# Autodesk Inventor assembly: Handle_ASAP3
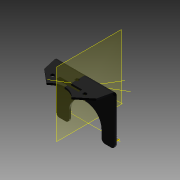
[picture p0: Inventor's stored thumbnail of the model, 180x180]
Saved by Autodesk Inventor 2011 SP2 (Build 150309200, 309)
## iProperties
Created: 2013-03-14
Part Number: Handle_ASAP3
Document SubType Name: Assembly
Designer: sungwook
Author: sungwook
## Documents named in this file (4)
- C:\Users\sungwook\Documents\Inventor\Micron22_top_adj_02082013\Parts\ASAP\Handle_ASAP3.iam
- C:\Users\sungwook\Documents\Inventor\Micron22_top_adj_02082013\Parts\ASAP\ASAP_Handle_Fixture_New3.ipt
- C:\Users\sungwook\Documents\Inventor\Micron22_top_adj_02082013\Parts\ASAP\LED2.ipt
- C:\Users\sungwook\Documents\Inventor\Micron22_top_adj_02082013\Parts\ASAP\LED2_MIR3.ipt
## Components (4 placed, 3 different names)
1. ASAP_Handle_Fixture_New3:1 — Mate:1, Mate:2, Mate:3, Mate:4, Mate:5, Mate:6
2. LED2:1 — Mate:1, Mate:2, Mate:3
3. LED2:2 — Mate:4, Mate:5, Mate:6
4. LED2_MIR3:1
## Relationships (6: Mate 6)
- Mate:1: ASAP_Handle_Fixture_New3:1 ↔ LED2:1
- Mate:2 (-2.25 mm): ASAP_Handle_Fixture_New3:1 ↔ LED2:1
- Mate:3 (-1.75 mm): ASAP_Handle_Fixture_New3:1 ↔ LED2:1
- Mate:4: ASAP_Handle_Fixture_New3:1 ↔ LED2:2
- Mate:5 (-13.25 mm): ASAP_Handle_Fixture_New3:1 ↔ LED2:2
- Mate:6 (-10 mm): ASAP_Handle_Fixture_New3:1 ↔ LED2:2
